# Autodesk Inventor assembly: Y Idler
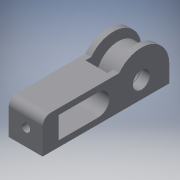
[picture p0: Inventor's stored thumbnail of the model, 180x180]
Saved by Autodesk Inventor 2018 (Build 220112000, 112)
## iProperties
Created: 2018-06-16
Part Number: Y Idler
Document SubType Name: Assembly
Designer: Jasper
Author: Jasper
## Documents named in this file (3)
- C:\Users\Jasper\Downloads\git_WSL\MEME_MACHINE\CAD\Y Idler\Y Idler.iam
- C:\Users\Jasper\Downloads\git_WSL\MEME_MACHINE\CAD\Y Idler\Y Idler.ipt
- C:\Users\Jasper\Downloads\git_WSL\MEME_MACHINE\CAD\Vitamins\608 Bearing.ipt
## Components (2 placed, 2 different names)
1. Y Idler:1 — Mate:1, Mate:2
2. 608 Bearing:1 — Mate:1, Mate:2
## Relationships (2: Mate 2)
- Mate:1: Y Idler:1 ↔ 608 Bearing:1
- Mate:2: Y Idler:1 ↔ 608 Bearing:1
